# Autodesk Inventor assembly: Assembly1
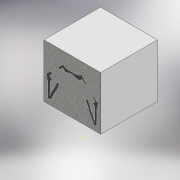
[picture p0: Inventor's stored thumbnail of the model, 180x180]
Saved by Autodesk Inventor 2021 (Build 250183000, 183)
## iProperties
Created: 2020-06-24
Part Number: Assembly1
Document SubType Name: Assembly
Designer: Derm
Author: Derm
## Documents named in this file (3)
- C:\Users\Derm\n95\v7\maskBodyV4Molds\Assembly1.iam
- C:\Users\Derm\n95\v7\maskBodyV4.ipt
- C:\Users\Derm\n95\v7\maskBodyV4Molds\mainMold.ipt
## Components (2 placed, 2 different names)
1. maskBodyV4:1 — Flush:1
2. mainMold:1 — Flush:1
## Relationships (1: Flush 1)
- Flush:1: maskBodyV4:1 ↔ mainMold:1
